# Autodesk Inventor assembly: колесо большое1 зеркальный
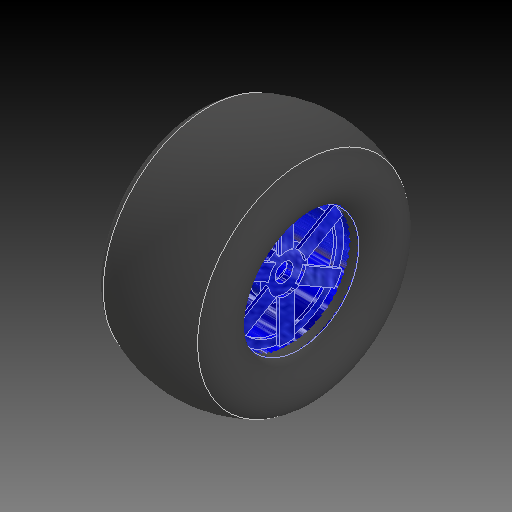
[picture p0: Inventor's stored thumbnail of the model, 512x512]
Saved by Autodesk Inventor 2020 (Build 240168000, 168)
## iProperties
Part Number: колесо большое1 зеркальный
Material: Типовые
Document SubType Name: Assembly
Designer: Петров Иван
Mass: 1000.36 g
Surface Area: 1140.53 cm^2
Volume: 1000.36 cm^3
Density: 1 g/cm^3
Author: sbnnl
## Documents named in this file (3)
- E:\IVAN\Ivan_desktop\Kvantorium\Projects\RoboPatrol\design\standart_components\WheelBig\колесо большое1 зеркальный.iam
- E:\IVAN\Ivan_desktop\Kvantorium\Projects\RoboPatrol\design\standart_components\WheelBig\шина1 зеркальный.ipt
- E:\IVAN\Ivan_desktop\Kvantorium\Projects\RoboPatrol\design\standart_components\WheelBig\диск1 зеркальный.ipt
## Components (2 placed, 2 different names)
1. шина1 зеркальный:1 — Совмещение:1
2. диск1 зеркальный:1 — Совмещение:1
## Relationships (1: Mate 1)
- Совмещение:1 [Mate]: шина1 зеркальный:1 ↔ диск1 зеркальный:1
